# Autodesk Inventor assembly: CapOnlyForWater
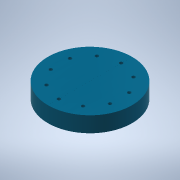
[picture p0: Inventor's stored thumbnail of the model, 180x180]
Saved by Autodesk Inventor 2021.1 (Build 251245000, 245)
## iProperties
Created: 2017-11-19
Part Number: CapOnlyForWater
Document SubType Name: Assembly
Designer: steele
Author: steele
## Documents named in this file (2)
- C:\git\CAD-Development\robSteele\HouseProjects\Garage\CapForWater\CapOnlyForWater.iam
- C:\git\CAD-Development\robSteele\HouseProjects\Garage\CapForWater\CoverPlateForWaterHalf.ipt
## Components (2 placed, 1 different names)
1. CoverPlateForWaterHalf:1 — Mate:1, Mate:2, Mate:3
2. CoverPlateForWaterHalf:2 — Mate:1, Mate:2, Mate:3
## Relationships (3: Mate 3)
- Mate:1: CoverPlateForWaterHalf:1 ↔ CoverPlateForWaterHalf:2
- Mate:2: CoverPlateForWaterHalf:1 ↔ CoverPlateForWaterHalf:2
- Mate:3: CoverPlateForWaterHalf:1 ↔ CoverPlateForWaterHalf:2
